# Autodesk Inventor assembly: Assembly6
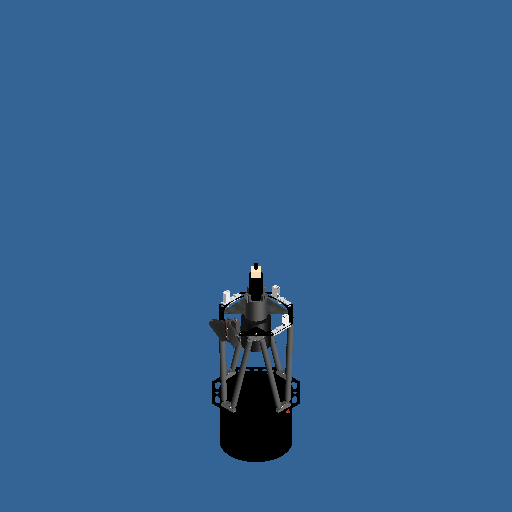
[picture p0: Inventor's stored thumbnail of the model, 512x512]
Saved by Autodesk Inventor 2026.2 (Build 302298000, 298)
## iProperties
Created: 2025-12-09
Part Number: Assembly6
Document SubType Name: Assembly
Designer: Thoma
Mass: 27295.5 g
Surface Area: 25498 cm^2
Volume: 10830.6 cm^3
Density: 2.52023 g/cm^3
Author: Thoma
## Documents named in this file (33)
- C:\Users\Thoma\OneDrive\Desktop\dir\telescope_cover\main\version_2\Main_v5.iam
- C:\Users\Thoma\OneDrive\Desktop\dir\telescope_cover\telescope\version_3\Telescope_End.ipt
- C:\Users\Thoma\OneDrive\Desktop\dir\telescope_cover\telescope\version_3\Triangle.ipt
- C:\Users\Thoma\OneDrive\Desktop\dir\telescope_cover\telescope\version_3\Triangle_Bracket_Top.ipt
- C:\Users\Thoma\OneDrive\Desktop\dir\telescope_cover\telescope\version_3\Carbon_Fibre.ipt
- C:\Users\Thoma\OneDrive\Desktop\dir\telescope_cover\telescope\version_3\5mm Screw.ipt
- C:\Users\Thoma\OneDrive\Desktop\dir\telescope_cover\telescope\version_3\35mm_bolt.ipt
- C:\Users\Thoma\OneDrive\Desktop\dir\telescope_cover\telescope\version_3\Triangle_Bracket_Bottom_MIR.ipt
- C:\Users\Thoma\OneDrive\Desktop\dir\telescope_cover\telescope\version_3\Telescope_Base.ipt
- C:\Users\Thoma\OneDrive\Desktop\dir\telescope_cover\telescope\version_3\Full_shaft_Simplify_3.ipt
- C:\Users\Thoma\OneDrive\Desktop\dir\telescope_cover\telescope\version_3\30mm_bolt.ipt
- C:\Users\Thoma\OneDrive\Desktop\dir\telescope_cover\telescope\version_3\Baffle.ipt
- C:\Users\Thoma\OneDrive\Desktop\dir\telescope_cover\telescope\version_3\Bottom_End_Top.ipt
- C:\Users\Thoma\OneDrive\Desktop\dir\telescope_cover\telescope\version_3\Laser.ipt
- C:\Users\Thoma\OneDrive\Desktop\dir\telescope_cover\cover\central_cover_v1.ipt
- C:\Users\Thoma\OneDrive\Desktop\dir\telescope_cover\cover\base_plate_v11.ipt
- C:\Users\Thoma\OneDrive\Desktop\dir\telescope_cover\cover\base_plate_bottom_v5.ipt
- C:\Users\Thoma\OneDrive\Documents\Inventor\Content Center Files\R2026\en-US\ISO 4035(2)\ISO 4035 - M4 - ISO.ipt
- C:\Users\Thoma\OneDrive\Desktop\dir\telescope_cover\servo\DSS-M15S Servo.ipt
- C:\Users\Thoma\OneDrive\Documents\Inventor\Content Center Files\R2026\en-US\ISO 4762(2)\ISO 4762 - M4 x 16ISO.ipt
- C:\Users\Thoma\OneDrive\Desktop\dir\telescope_cover\cover\pawn_v3.ipt
- C:\Users\Thoma\OneDrive\Documents\Inventor\Content Center Files\R2026\en-US\DIN 6796\DIN 6796 - 2.ipt
- C:\Users\Thoma\OneDrive\Documents\Inventor\Content Center Files\R2026\en-US\DIN 912\DIN 912 - M2 x 0.4 x 8 x 7.ipt
- C:\Users\Thoma\OneDrive\Documents\Inventor\Content Center Files\R2026\en-US\DIN 912\DIN 912 - M2 x 0.4 x 5 x 4.ipt
- C:\Users\Thoma\OneDrive\Desktop\dir\telescope_cover\cover\rod_v11.ipt
- C:\Users\Thoma\OneDrive\Documents\Inventor\Content Center Files\R2026\en-US\ISO 7092\ISO 7092 - ST 4 - 140 HV.ipt
- C:\Users\Thoma\OneDrive\Desktop\dir\telescope_cover\cover\Cover_Upper_v5.ipt
- C:\Users\Thoma\OneDrive\Desktop\dir\telescope_cover\cover\4mm_washer_1mm.ipt
- C:\Users\Thoma\OneDrive\Documents\Inventor\Content Center Files\R2026\en-US\ISO 4762(2)\ISO 4762 - M4 x 20ISO.ipt
- C:\Users\Thoma\OneDrive\Documents\Inventor\Content Center Files\R2026\en-US\ISO 4032(2)\ISO 4032 - M4 - ISO.ipt
- C:\Users\Thoma\OneDrive\Documents\Inventor\Content Center Files\R2026\en-US\ISO 7093 A\ISO 7093 A - ST 4 - 140 HV .ipt
- C:\Users\Thoma\OneDrive\Documents\Inventor\Content Center Files\R2026\en-US\ISO 4762(2)\ISO 4762 - M4 x 30ISO.ipt
- C:\Users\Thoma\OneDrive\Desktop\dir\telescope_cover\servo\limit_switch_v2.ipt
## Components (119 placed, 32 different names)
1. base_plate_bottom_v5:2 — Mate:332, Mate:333, Mate:334, Mate:353, Mate:357, Mate:361
2. base_plate_v11:2 — Mate:341, Mate:344, Mate:345
3. base_plate_bottom_v5:3 — Mate:338, Mate:339, Mate:340
4. base_plate_v11:3 — Mate:343, Mate:348, Mate:349, Mate:350, Mate:351, Mate:352, Mate:354, Mate:355, Mate:356, Mate:358, Mate:359, Mate:360
5. base_plate_bottom_v5:4 — Mate:335, Mate:336, Mate:337
6. base_plate_v11:4 — Mate:342, Mate:346, Mate:347
7. ISO 7092 ST 4 - 140 HV:14 — Mate:350, Mate:351, Insert:26
8. ISO 4762 M4 x 30:2 — Insert:26
9. ISO 7093 A ST 4 - 140 HV - A:4 — Mate:352, Mate:353, Insert:27
10. ISO 4032 M4:5 — Insert:27
11. ISO 7092 ST 4 - 140 HV:15 — Mate:354, Mate:355, Insert:28
12. ISO 4762 M4 x 20:6 — Insert:28
13. ISO 7093 A ST 4 - 140 HV - A:5 — Mate:356, Mate:357, Insert:29
14. ISO 4032 M4:6 — Insert:29
15. ISO 7092 ST 4 - 140 HV:16 — Mate:358, Mate:359, Insert:30
16. ISO 4762 M4 x 20:7 — Insert:30
17. ISO 7093 A ST 4 - 140 HV - A:6 — Mate:360, Mate:361, Insert:31
18. ISO 4032 M4:7 — Insert:31
19. base_plate_bottom_v5:5 — Mate:362, Mate:363, Mate:364, Mate:370, Mate:371, Flush:227
20. limit_switch_v2:1 — Mate:367, Mate:368, Mate:369
21. limit_switch_v2:2 — Mate:370, Mate:371, Flush:227
22. Laser:2 — Mate:214, Flush:220, Flush:221
23. Laser:1 — Mate:215, Flush:218, Flush:219
24. Baffle:1 — Mate:83
25. Carbon_Fibre:1 — Mate:7, Mate:11, Flush:1, Mate:12, Mate:13, Mate:14, Mate:15, Mate:62, Mate:83, Mate:92, Mate:93, Mate:96, Mate:97, Mate:98, Mate:100, Mate:123, Mate:124, Mate:125, Mate:213, Mate:220, Angle:84, Flush:223, Flush:224, Flush:225, Flush:226
26. Telescope_Base:1 — Mate:62, Angle:31, Mate:89, Mate:90, Angle:40, Mate:108, Mate:109, Angle:48, Mate:110, Mate:111, Angle:49, Mate:112, Mate:113, Angle:50, Mate:214, Mate:215, Flush:218, Flush:221
27. Telescope_End:1 — Mate:1, Mate:2, Angle:2, Mate:7, Mate:54, Mate:55, Angle:26, Angle:31, Mate:86, Mate:88, Mate:91, Angle:41, Mate:101, Angle:45, Angle:46, Mate:114, Mate:115, Angle:51, Mate:116, Mate:117, Angle:52, Mate:118, Mate:119, Angle:53, Mate:229, Angle:85, Mate:230, Mate:231, Mate:332, Mate:333, Mate:334, Mate:335, Mate:336, Mate:337, Mate:338, Mate:339, Mate:340, Mate:341, Mate:342, Mate:343, Mate:344, Mate:345, Mate:346, Mate:347, Mate:348, Mate:349, Mate:362
28. 30mm_bolt:9 — Mate:217, Mate:218, Angle:83
29. 30mm_bolt:10 — Mate:216, Mate:219, Angle:82
30. Triangle_Bracket_Top:5 — Mate:116, Mate:117, Angle:52, Mate:129, Flush:110, Angle:60
31. Triangle_Bracket_Top:4 — Mate:101, Angle:45, Angle:46, Mate:104, Mate:105, Mate:106, Flush:103, Angle:47
32. Triangle_Bracket_Top:3 — Mate:86, Mate:88, Mate:94, Angle:54, Angle:55, Mate:122, Flush:106, Angle:56
33. Triangle_Bracket_Top:1 — Mate:1, Mate:2, Angle:2, Mate:8, Mate:9, Angle:4, Mate:47, Angle:22, Mate:58
34. 5mm Screw:14 — Mate:220, Flush:222, Angle:84
35. Triangle:1 — Mate:8, Mate:9, Angle:4, Mate:11, Flush:1, Angle:5, Angle:6, Mate:46, Mate:222, Mate:223
36. Triangle:5 — Mate:92, Mate:93, Mate:94, Mate:128, Flush:109, Angle:59, Flush:181, Angle:81, Mate:225, Mate:227
37. Triangle:6 — Mate:96, Mate:97, Mate:98, Flush:102, Angle:44, Mate:104, Mate:105, Flush:222, Mate:221, Mate:228
38. Triangle:7 — Mate:123, Mate:124, Mate:125, Mate:126, Flush:107, Angle:57, Mate:127, Flush:108, Angle:58, Mate:224, Mate:226
39. 35mm_bolt:6 — Mate:122, Flush:106, Angle:56
40. 35mm_bolt:7 — Mate:129, Flush:110, Angle:60
41. 35mm_bolt:4 — Mate:46, Mate:47, Angle:22
42. 35mm_bolt:5 — Mate:106, Flush:103, Angle:47
43. 5mm Screw:9 — Mate:100, Flush:102, Angle:44
44. 5mm Screw:13 — Mate:213, Flush:181, Angle:81
45. 5mm Screw:10 — Mate:126, Flush:107, Angle:57
46. 5mm Screw:2 — Mate:14, Mate:15, Angle:6
47. 5mm Screw:1 — Mate:12, Mate:13, Angle:5
48. 5mm Screw:11 — Mate:127, Flush:108, Angle:58
49. 5mm Screw:12 — Mate:128, Flush:109, Angle:59
50. Full_shaft_Simplify_3:1
51. Full_shaft_Simplify_3:2 — Tangent:26
52. Full_shaft_Simplify_3:3
53. Full_shaft_Simplify_3:4
54. Full_shaft_Simplify_3:5
55. Full_shaft_Simplify_3:6
56. Full_shaft_Simplify_3:7
57. Full_shaft_Simplify_3:8 — Tangent:31, Tangent:33
58. 30mm_bolt:7 — Mate:120, Flush:104, Angle:54
59. 30mm_bolt:1 — Mate:121, Flush:105, Angle:55
60. 30mm_bolt:8 — Mate:80, Flush:13, Angle:39
61. 30mm_bolt:6 — Mate:78, Flush:11, Angle:37
62. 30mm_bolt:3 — Mate:79, Flush:12, Angle:38
63. 30mm_bolt:2 — Mate:77, Flush:10, Angle:36
64. Triangle_Bracket_Bottom_MIR:4 — Mate:118, Mate:119, Angle:53, Mate:216, Mate:217, Mate:218, Mate:219, Angle:82, Angle:83
65. Triangle_Bracket_Bottom_MIR:3 — Mate:114, Mate:115, Angle:51, Mate:120, Flush:104, Mate:121, Flush:105
66. Triangle_Bracket_Bottom_MIR:2 — Mate:55, Mate:58, Angle:26, Mate:77, Flush:10, Angle:36, Mate:78, Flush:11, Angle:37, Tangent:31
67. Triangle_Bracket_Bottom_MIR:1 — Mate:54, Mate:79, Flush:12, Angle:38, Mate:80, Flush:13, Angle:39, Mate:91, Angle:41
68. Bottom_End_Top:4 — Mate:112, Mate:113, Angle:50, Tangent:26, Tangent:33
69. Bottom_End_Top:3 — Mate:110, Mate:111, Angle:49, Flush:219
70. Bottom_End_Top:2 — Mate:108, Mate:109, Angle:48
71. Bottom_End_Top:1 — Mate:89, Mate:90, Angle:40, Flush:220
72. central_cover_v1:1 — Mate:221, Mate:222, Flush:223, Mate:367, Mate:368, Mate:369
73. central_cover_v1:2 — Mate:223, Mate:224, Flush:224
74. central_cover_v1:3 — Mate:225, Mate:226, Flush:225
75. central_cover_v1:4 — Mate:227, Mate:228, Flush:226
76. base_plate_v11:1 — Mate:229, Angle:85, Mate:230, Mate:231, Angle:92, Mate:262, Mate:263, Mate:264, Mate:271, Mate:272, Mate:273, Mate:274, Mate:275, Mate:276, Mate:277, Mate:278, Mate:282, Mate:307, Mate:308, Mate:309, Mate:310, Mate:312, Mate:314, Mate:320, Mate:321, Mate:322, Mate:324, Mate:325, Mate:326, Mate:328, Mate:329, Mate:330
77. pawn_v3:1 — Angle:92, Mate:281, Mate:282, Mate:311, Mate:313
78. DSS-M15S Servo:1 — Mate:262, Mate:263, Mate:264, Mate:279, Mate:280
79. DIN 6796 2:1 — Mate:271, Mate:272, Insert:6
80. DIN 912 - replaced by DIN EN ISO 4762 M2 x 8:1 — Insert:6
81. DIN 6796 2:2 — Mate:273, Mate:274, Insert:7
82. DIN 912 - replaced by DIN EN ISO 4762 M2 x 5:1 — Insert:7
83. DIN 6796 2:3 — Mate:275, Mate:276, Insert:8
84. DIN 912 - replaced by DIN EN ISO 4762 M2 x 8:2 — Insert:8
85. DIN 6796 2:4 — Mate:277, Mate:278, Insert:9
86. DIN 912 - replaced by DIN EN ISO 4762 M2 x 8:3 — Insert:9
87. rod_v11:1 — Mate:279, Mate:280, Mate:281, Mate:287, Mate:288, Tangent:34, Mate:289, Mate:290, Mate:291, Mate:292, Mate:293, Mate:294, Mate:295, Mate:297, Mate:298, Mate:299, Mate:301, Mate:302, Mate:303, Mate:305, Mate:306
88. Cover_Upper_v5:1 — Mate:287, Mate:288, Tangent:34, Mate:296, Mate:300, Mate:304
89. 4mm_washer_1mm:1 — Mate:289, Mate:294
90. 4mm_washer_1mm:2 — Mate:290, Mate:293
91. 4mm_washer_1mm:3 — Mate:291, Mate:292
92. ISO 7092 ST 4 - 140 HV:3 — Mate:295, Mate:296, Insert:12
93. ISO 4762 M4 x 16:3 — Insert:12
94. ISO 7092 ST 4 - 140 HV:4 — Mate:297, Mate:298, Insert:13
95. ISO 4035 M4:5 — Insert:13
96. ISO 7092 ST 4 - 140 HV:5 — Mate:299, Mate:300, Insert:14
97. ISO 4762 M4 x 16:4 — Insert:14
98. ISO 7092 ST 4 - 140 HV:6 — Mate:301, Mate:302, Insert:15
99. ISO 4035 M4:6 — Insert:15
100. ISO 7092 ST 4 - 140 HV:7 — Mate:303, Mate:304, Insert:16
101. ISO 4762 M4 x 16:5 — Insert:16
102. ISO 7092 ST 4 - 140 HV:8 — Mate:305, Mate:306, Insert:17
103. ISO 4035 M4:7 — Insert:17
104. ISO 4762 M4 x 20:1 — Mate:307, Mate:308
105. ISO 4035 M4:8 — Mate:309, Mate:310
106. ISO 4762 M4 x 20:2 — Mate:311, Mate:312
107. ISO 4035 M4:9 — Mate:313, Mate:314
108. ISO 7092 ST 4 - 140 HV:11 — Mate:320, Mate:321, Insert:20
109. ISO 4762 M4 x 20:4 — Insert:20
110. ISO 7093 A ST 4 - 140 HV - A:1 — Mate:322, Insert:21
111. ISO 4032 M4:2 — Insert:21
112. ISO 7092 ST 4 - 140 HV:12 — Mate:324, Mate:325, Insert:22
113. ISO 4762 M4 x 20:5 — Insert:22, Mate:363
114. ISO 7093 A ST 4 - 140 HV - A:2 — Mate:326, Insert:23
115. ISO 4032 M4:3 — Insert:23
116. ISO 7092 ST 4 - 140 HV:13 — Mate:328, Mate:329, Insert:24
117. ISO 4762 M4 x 30:1 — Insert:24, Mate:364
118. ISO 7093 A ST 4 - 140 HV - A:3 — Mate:330, Insert:25
119. ISO 4032 M4:4 — Insert:25
## Relationships (255: Mate 168, Angle 36, Flush 25, Insert 22, Tangent 4)
- Mate:1: Telescope_End:1 ↔ Triangle_Bracket_Top:1
- Mate:2: Telescope_End:1 ↔ Triangle_Bracket_Top:1
- Angle:2 (0 deg): Telescope_End:1 ↔ Triangle_Bracket_Top:1
- Mate:7: Carbon_Fibre:1 ↔ Telescope_End:1
- Mate:8: Triangle_Bracket_Top:1 ↔ Triangle:1
- Mate:9: Triangle_Bracket_Top:1 ↔ Triangle:1
- Angle:4 (0 deg): Triangle_Bracket_Top:1 ↔ Triangle:1
- Mate:11: Carbon_Fibre:1 ↔ Triangle:1
- Flush:1: Carbon_Fibre:1 ↔ Triangle:1
- Mate:12: Carbon_Fibre:1 ↔ 5mm Screw:1
- Mate:13: Carbon_Fibre:1 ↔ 5mm Screw:1
- Angle:5 (0 deg): Triangle:1 ↔ 5mm Screw:1
- Mate:14: Carbon_Fibre:1 ↔ 5mm Screw:2
- Mate:15: Carbon_Fibre:1 ↔ 5mm Screw:2
- Angle:6 (0 deg): Triangle:1 ↔ 5mm Screw:2
- Mate:46: Triangle:1 ↔ 35mm_bolt:4
- Mate:47: Triangle_Bracket_Top:1 ↔ 35mm_bolt:4
- Angle:22 (0 deg): Triangle_Bracket_Top:1 ↔ 35mm_bolt:4
- Mate:54: Telescope_End:1 ↔ Triangle_Bracket_Bottom_MIR:1
- Mate:55: Telescope_End:1 ↔ Triangle_Bracket_Bottom_MIR:2
- Mate:58: Triangle_Bracket_Top:1 ↔ Triangle_Bracket_Bottom_MIR:2
- Angle:26 (0 deg): Telescope_End:1 ↔ Triangle_Bracket_Bottom_MIR:2
- Mate:62: Carbon_Fibre:1 ↔ Telescope_Base:1
- Angle:31 (0 deg): Telescope_Base:1 ↔ Telescope_End:1
- Mate:77: 30mm_bolt:2 ↔ Triangle_Bracket_Bottom_MIR:2
- Flush:10: 30mm_bolt:2 ↔ Triangle_Bracket_Bottom_MIR:2
- Angle:36 (0 deg): 30mm_bolt:2 ↔ Triangle_Bracket_Bottom_MIR:2
- Mate:78: 30mm_bolt:6 ↔ Triangle_Bracket_Bottom_MIR:2
- Flush:11: 30mm_bolt:6 ↔ Triangle_Bracket_Bottom_MIR:2
- Angle:37 (0 deg): 30mm_bolt:6 ↔ Triangle_Bracket_Bottom_MIR:2
- Mate:79: 30mm_bolt:3 ↔ Triangle_Bracket_Bottom_MIR:1
- Flush:12: 30mm_bolt:3 ↔ Triangle_Bracket_Bottom_MIR:1
- Angle:38 (0 deg): 30mm_bolt:3 ↔ Triangle_Bracket_Bottom_MIR:1
- Mate:80: 30mm_bolt:8 ↔ Triangle_Bracket_Bottom_MIR:1
- Flush:13: 30mm_bolt:8 ↔ Triangle_Bracket_Bottom_MIR:1
- Angle:39 (0 deg): 30mm_bolt:8 ↔ Triangle_Bracket_Bottom_MIR:1
- Mate:83: Baffle:1 ↔ Carbon_Fibre:1
- Mate:86: Telescope_End:1 ↔ Triangle_Bracket_Top:3
- Mate:88: Telescope_End:1 ↔ Triangle_Bracket_Top:3
- Mate:89: Telescope_Base:1 ↔ Bottom_End_Top:1
- Mate:90: Telescope_Base:1 ↔ Bottom_End_Top:1
- Angle:40 (0 deg): Telescope_Base:1 ↔ Bottom_End_Top:1
- Mate:91: Telescope_End:1 ↔ Triangle_Bracket_Bottom_MIR:1
- Angle:41 (0 deg): Telescope_End:1 ↔ Triangle_Bracket_Bottom_MIR:1
- Mate:92: Carbon_Fibre:1 ↔ Triangle:5
- Mate:93: Carbon_Fibre:1 ↔ Triangle:5
- Mate:94: Triangle_Bracket_Top:3 ↔ Triangle:5
- Mate:96: Carbon_Fibre:1 ↔ Triangle:6
- Mate:97: Carbon_Fibre:1 ↔ Triangle:6
- Mate:98: Carbon_Fibre:1 ↔ Triangle:6
- Mate:100: Carbon_Fibre:1 ↔ 5mm Screw:9
- Flush:102: Triangle:6 ↔ 5mm Screw:9
- Angle:44 (0 deg): Triangle:6 ↔ 5mm Screw:9
- Mate:101: Telescope_End:1 ↔ Triangle_Bracket_Top:4
- Angle:45 (0 deg): Telescope_End:1 ↔ Triangle_Bracket_Top:4
- Angle:46 (0 deg): Telescope_End:1 ↔ Triangle_Bracket_Top:4
- Mate:104: Triangle_Bracket_Top:4 ↔ Triangle:6
- Mate:105: Triangle_Bracket_Top:4 ↔ Triangle:6
- Mate:106: Triangle_Bracket_Top:4 ↔ 35mm_bolt:5
- Flush:103: Triangle_Bracket_Top:4 ↔ 35mm_bolt:5
- Angle:47 (0 deg): Triangle_Bracket_Top:4 ↔ 35mm_bolt:5
- Mate:108: Telescope_Base:1 ↔ Bottom_End_Top:2
- Mate:109: Telescope_Base:1 ↔ Bottom_End_Top:2
- Angle:48 (0 deg): Telescope_Base:1 ↔ Bottom_End_Top:2
- Mate:110: Telescope_Base:1 ↔ Bottom_End_Top:3
- Mate:111: Telescope_Base:1 ↔ Bottom_End_Top:3
- Angle:49 (0 deg): Telescope_Base:1 ↔ Bottom_End_Top:3
- Mate:112: Telescope_Base:1 ↔ Bottom_End_Top:4
- Mate:113: Telescope_Base:1 ↔ Bottom_End_Top:4
- Angle:50 (0 deg): Telescope_Base:1 ↔ Bottom_End_Top:4
- Mate:114: Telescope_End:1 ↔ Triangle_Bracket_Bottom_MIR:3
- Mate:115: Telescope_End:1 ↔ Triangle_Bracket_Bottom_MIR:3
- Angle:51 (0 deg): Telescope_End:1 ↔ Triangle_Bracket_Bottom_MIR:3
- Mate:116: Telescope_End:1 ↔ Triangle_Bracket_Top:5
- Mate:117: Telescope_End:1 ↔ Triangle_Bracket_Top:5
- Angle:52 (0 deg): Telescope_End:1 ↔ Triangle_Bracket_Top:5
- Mate:118: Telescope_End:1 ↔ Triangle_Bracket_Bottom_MIR:4
- Mate:119: Telescope_End:1 ↔ Triangle_Bracket_Bottom_MIR:4
- Angle:53 (0 deg): Telescope_End:1 ↔ Triangle_Bracket_Bottom_MIR:4
- Mate:120: 30mm_bolt:7 ↔ Triangle_Bracket_Bottom_MIR:3
- Flush:104: 30mm_bolt:7 ↔ Triangle_Bracket_Bottom_MIR:3
- Angle:54 (0 deg): Triangle_Bracket_Top:3 ↔ 30mm_bolt:7
- Mate:121: 30mm_bolt:1 ↔ Triangle_Bracket_Bottom_MIR:3
- Flush:105: 30mm_bolt:1 ↔ Triangle_Bracket_Bottom_MIR:3
- Angle:55 (0 deg): Triangle_Bracket_Top:3 ↔ 30mm_bolt:1
- Mate:122: Triangle_Bracket_Top:3 ↔ 35mm_bolt:6
- Flush:106: Triangle_Bracket_Top:3 ↔ 35mm_bolt:6
- Angle:56 (0 deg): Triangle_Bracket_Top:3 ↔ 35mm_bolt:6
- Mate:123: Carbon_Fibre:1 ↔ Triangle:7
- Mate:124: Carbon_Fibre:1 ↔ Triangle:7
- Mate:125: Carbon_Fibre:1 ↔ Triangle:7
- Mate:126: Triangle:7 ↔ 5mm Screw:10
- Flush:107: Triangle:7 ↔ 5mm Screw:10
- Angle:57 (0 deg): Triangle:7 ↔ 5mm Screw:10
- Mate:127: Triangle:7 ↔ 5mm Screw:11
- Flush:108: Triangle:7 ↔ 5mm Screw:11
- Angle:58 (0 deg): Triangle:7 ↔ 5mm Screw:11
- Mate:128: Triangle:5 ↔ 5mm Screw:12
- Flush:109: Triangle:5 ↔ 5mm Screw:12
- Angle:59 (0 deg): Triangle:5 ↔ 5mm Screw:12
- Mate:129: Triangle_Bracket_Top:5 ↔ 35mm_bolt:7
- Flush:110: Triangle_Bracket_Top:5 ↔ 35mm_bolt:7
- Angle:60 (0 deg): Triangle_Bracket_Top:5 ↔ 35mm_bolt:7
- Mate:213: Carbon_Fibre:1 ↔ 5mm Screw:13
- Flush:181: Triangle:5 ↔ 5mm Screw:13
- Angle:81 (0 deg): Triangle:5 ↔ 5mm Screw:13
- Mate:214: Laser:2 ↔ Telescope_Base:1
- Mate:215: Laser:1 ↔ Telescope_Base:1
- Flush:218: Laser:1 ↔ Telescope_Base:1
- Flush:219 (39.316 mm): Laser:1 ↔ Bottom_End_Top:3
- Flush:220 (39.316 mm): Laser:2 ↔ Bottom_End_Top:1
- Flush:221: Laser:2 ↔ Telescope_Base:1
- Tangent:26: Full_shaft_Simplify_3:2 ↔ Bottom_End_Top:4
- Tangent:31: Full_shaft_Simplify_3:8 ↔ Triangle_Bracket_Bottom_MIR:2
- Tangent:33: Full_shaft_Simplify_3:8 ↔ Bottom_End_Top:4
- Mate:216: 30mm_bolt:10 ↔ Triangle_Bracket_Bottom_MIR:4
- Mate:217: 30mm_bolt:9 ↔ Triangle_Bracket_Bottom_MIR:4
- Mate:218: 30mm_bolt:9 ↔ Triangle_Bracket_Bottom_MIR:4
- Mate:219: 30mm_bolt:10 ↔ Triangle_Bracket_Bottom_MIR:4
- Angle:82 (0 deg): 30mm_bolt:10 ↔ Triangle_Bracket_Bottom_MIR:4
- Angle:83 (0 deg): 30mm_bolt:9 ↔ Triangle_Bracket_Bottom_MIR:4
- Mate:220: Carbon_Fibre:1 ↔ 5mm Screw:14
- Flush:222: 5mm Screw:14 ↔ Triangle:6
- Angle:84 (0 deg): Carbon_Fibre:1 ↔ 5mm Screw:14
- Mate:221: Triangle:6 ↔ central_cover_v1:1
- Mate:222: Triangle:1 ↔ central_cover_v1:1
- Flush:223: Carbon_Fibre:1 ↔ central_cover_v1:1
- Mate:223: Triangle:1 ↔ central_cover_v1:2
- Mate:224: Triangle:7 ↔ central_cover_v1:2
- Flush:224: Carbon_Fibre:1 ↔ central_cover_v1:2
- Mate:225: Triangle:5 ↔ central_cover_v1:3
- Mate:226: Triangle:7 ↔ central_cover_v1:3
- Flush:225: Carbon_Fibre:1 ↔ central_cover_v1:3
- Mate:227: Triangle:5 ↔ central_cover_v1:4
- Mate:228: Triangle:6 ↔ central_cover_v1:4
- Flush:226: Carbon_Fibre:1 ↔ central_cover_v1:4
- Mate:229: Telescope_End:1 ↔ base_plate_v11:1
- Angle:85 (0 deg): Telescope_End:1 ↔ base_plate_v11:1
- Mate:230: Telescope_End:1 ↔ base_plate_v11:1
- Mate:231: Telescope_End:1 ↔ base_plate_v11:1
- Angle:92 (0 deg): base_plate_v11:1 ↔ pawn_v3:1
- Mate:262: base_plate_v11:1 ↔ DSS-M15S Servo:1
- Mate:263 (1.1 mm): base_plate_v11:1 ↔ DSS-M15S Servo:1
- Mate:264: base_plate_v11:1 ↔ DSS-M15S Servo:1
- Mate:271: base_plate_v11:1 ↔ DIN 6796 2:1
- Mate:272: base_plate_v11:1 ↔ DIN 6796 2:1
- Insert:6: DIN 6796 2:1 ↔ DIN 912 - replaced by DIN EN ISO 4762 M2 x 8:1
- Mate:273: base_plate_v11:1 ↔ DIN 6796 2:2
- Mate:274: base_plate_v11:1 ↔ DIN 6796 2:2
- Insert:7: DIN 6796 2:2 ↔ DIN 912 - replaced by DIN EN ISO 4762 M2 x 5:1
- Mate:275: base_plate_v11:1 ↔ DIN 6796 2:3
- Mate:276: base_plate_v11:1 ↔ DIN 6796 2:3
- Insert:8: DIN 6796 2:3 ↔ DIN 912 - replaced by DIN EN ISO 4762 M2 x 8:2
- Mate:277: base_plate_v11:1 ↔ DIN 6796 2:4
- Mate:278: base_plate_v11:1 ↔ DIN 6796 2:4
- Insert:9: DIN 6796 2:4 ↔ DIN 912 - replaced by DIN EN ISO 4762 M2 x 8:3
- Mate:279: DSS-M15S Servo:1 ↔ rod_v11:1
- Mate:280: DSS-M15S Servo:1 ↔ rod_v11:1
- Mate:281: pawn_v3:1 ↔ rod_v11:1
- Mate:282 (0.4 mm): base_plate_v11:1 ↔ pawn_v3:1
- Mate:287: rod_v11:1 ↔ Cover_Upper_v5:1
- Mate:288: rod_v11:1 ↔ Cover_Upper_v5:1
- Tangent:34 (-1 mm): rod_v11:1 ↔ Cover_Upper_v5:1
- Mate:289: rod_v11:1 ↔ 4mm_washer_1mm:1
- Mate:290: rod_v11:1 ↔ 4mm_washer_1mm:2
- Mate:291: rod_v11:1 ↔ 4mm_washer_1mm:3
- Mate:292: rod_v11:1 ↔ 4mm_washer_1mm:3
- Mate:293: rod_v11:1 ↔ 4mm_washer_1mm:2
- Mate:294: rod_v11:1 ↔ 4mm_washer_1mm:1
- Mate:295: rod_v11:1 ↔ ISO 7092 ST 4 - 140 HV:3
- Mate:296: Cover_Upper_v5:1 ↔ ISO 7092 ST 4 - 140 HV:3
- Insert:12: ISO 7092 ST 4 - 140 HV:3 ↔ ISO 4762 M4 x 16:3
- Mate:297: rod_v11:1 ↔ ISO 7092 ST 4 - 140 HV:4
- Mate:298: rod_v11:1 ↔ ISO 7092 ST 4 - 140 HV:4
- Insert:13: ISO 7092 ST 4 - 140 HV:4 ↔ ISO 4035 M4:5
- Mate:299: rod_v11:1 ↔ ISO 7092 ST 4 - 140 HV:5
- Mate:300: Cover_Upper_v5:1 ↔ ISO 7092 ST 4 - 140 HV:5
- Insert:14: ISO 7092 ST 4 - 140 HV:5 ↔ ISO 4762 M4 x 16:4
- Mate:301: rod_v11:1 ↔ ISO 7092 ST 4 - 140 HV:6
- Mate:302: rod_v11:1 ↔ ISO 7092 ST 4 - 140 HV:6
- Insert:15: ISO 7092 ST 4 - 140 HV:6 ↔ ISO 4035 M4:6
- Mate:303: rod_v11:1 ↔ ISO 7092 ST 4 - 140 HV:7
- Mate:304: Cover_Upper_v5:1 ↔ ISO 7092 ST 4 - 140 HV:7
- Insert:16: ISO 7092 ST 4 - 140 HV:7 ↔ ISO 4762 M4 x 16:5
- Mate:305: rod_v11:1 ↔ ISO 7092 ST 4 - 140 HV:8
- Mate:306: rod_v11:1 ↔ ISO 7092 ST 4 - 140 HV:8
- Insert:17: ISO 7092 ST 4 - 140 HV:8 ↔ ISO 4035 M4:7
- Mate:307: base_plate_v11:1 ↔ ISO 4762 M4 x 20:1
- Mate:308: base_plate_v11:1 ↔ ISO 4762 M4 x 20:1
- Mate:309: base_plate_v11:1 ↔ ISO 4035 M4:8
- Mate:310: base_plate_v11:1 ↔ ISO 4035 M4:8
- Mate:311: pawn_v3:1 ↔ ISO 4762 M4 x 20:2
- Mate:312: base_plate_v11:1 ↔ ISO 4762 M4 x 20:2
- Mate:313: pawn_v3:1 ↔ ISO 4035 M4:9
- Mate:314: base_plate_v11:1 ↔ ISO 4035 M4:9
- Mate:320: base_plate_v11:1 ↔ ISO 7092 ST 4 - 140 HV:11
- Mate:321: base_plate_v11:1 ↔ ISO 7092 ST 4 - 140 HV:11
- Insert:20: ISO 7092 ST 4 - 140 HV:11 ↔ ISO 4762 M4 x 20:4
- Mate:322: base_plate_v11:1 ↔ ISO 7093 A ST 4 - 140 HV - A:1
- Insert:21: ISO 7093 A ST 4 - 140 HV - A:1 ↔ ISO 4032 M4:2
- Mate:324: base_plate_v11:1 ↔ ISO 7092 ST 4 - 140 HV:12
- Mate:325: base_plate_v11:1 ↔ ISO 7092 ST 4 - 140 HV:12
- Insert:22: ISO 7092 ST 4 - 140 HV:12 ↔ ISO 4762 M4 x 20:5
- Mate:326: base_plate_v11:1 ↔ ISO 7093 A ST 4 - 140 HV - A:2
- Insert:23: ISO 7093 A ST 4 - 140 HV - A:2 ↔ ISO 4032 M4:3
- Mate:328: base_plate_v11:1 ↔ ISO 7092 ST 4 - 140 HV:13
- Mate:329: base_plate_v11:1 ↔ ISO 7092 ST 4 - 140 HV:13
- Insert:24: ISO 7092 ST 4 - 140 HV:13 ↔ ISO 4762 M4 x 30:1
- Mate:330: base_plate_v11:1 ↔ ISO 7093 A ST 4 - 140 HV - A:3
- Insert:25: ISO 7093 A ST 4 - 140 HV - A:3 ↔ ISO 4032 M4:4
- Mate:332: base_plate_bottom_v5:2 ↔ Telescope_End:1
- Mate:333: base_plate_bottom_v5:2 ↔ Telescope_End:1
- Mate:334: base_plate_bottom_v5:2 ↔ Telescope_End:1
- Mate:335: base_plate_bottom_v5:4 ↔ Telescope_End:1
- Mate:336: base_plate_bottom_v5:4 ↔ Telescope_End:1
- Mate:337: base_plate_bottom_v5:4 ↔ Telescope_End:1
- Mate:338: base_plate_bottom_v5:3 ↔ Telescope_End:1
- Mate:339: base_plate_bottom_v5:3 ↔ Telescope_End:1
- Mate:340: base_plate_bottom_v5:3 ↔ Telescope_End:1
- Mate:341: base_plate_v11:2 ↔ Telescope_End:1
- Mate:342: base_plate_v11:4 ↔ Telescope_End:1
- Mate:343: base_plate_v11:3 ↔ Telescope_End:1
- Mate:344: base_plate_v11:2 ↔ Telescope_End:1
- Mate:345: base_plate_v11:2 ↔ Telescope_End:1
- Mate:346: base_plate_v11:4 ↔ Telescope_End:1
- Mate:347: base_plate_v11:4 ↔ Telescope_End:1
- Mate:348: base_plate_v11:3 ↔ Telescope_End:1
- Mate:349: base_plate_v11:3 ↔ Telescope_End:1
- Mate:350: base_plate_v11:3 ↔ ISO 7092 ST 4 - 140 HV:14
- Mate:351: base_plate_v11:3 ↔ ISO 7092 ST 4 - 140 HV:14
- Insert:26: ISO 7092 ST 4 - 140 HV:14 ↔ ISO 4762 M4 x 30:2
- Mate:352: base_plate_v11:3 ↔ ISO 7093 A ST 4 - 140 HV - A:4
- Mate:353: base_plate_bottom_v5:2 ↔ ISO 7093 A ST 4 - 140 HV - A:4
- Insert:27: ISO 7093 A ST 4 - 140 HV - A:4 ↔ ISO 4032 M4:5
- Mate:354: base_plate_v11:3 ↔ ISO 7092 ST 4 - 140 HV:15
- Mate:355: base_plate_v11:3 ↔ ISO 7092 ST 4 - 140 HV:15
- Insert:28: ISO 7092 ST 4 - 140 HV:15 ↔ ISO 4762 M4 x 20:6
- Mate:356: base_plate_v11:3 ↔ ISO 7093 A ST 4 - 140 HV - A:5
- Mate:357: base_plate_bottom_v5:2 ↔ ISO 7093 A ST 4 - 140 HV - A:5
- Insert:29: ISO 7093 A ST 4 - 140 HV - A:5 ↔ ISO 4032 M4:6
- Mate:358: base_plate_v11:3 ↔ ISO 7092 ST 4 - 140 HV:16
- Mate:359: base_plate_v11:3 ↔ ISO 7092 ST 4 - 140 HV:16
- Insert:30: ISO 7092 ST 4 - 140 HV:16 ↔ ISO 4762 M4 x 20:7
- Mate:360: base_plate_v11:3 ↔ ISO 7093 A ST 4 - 140 HV - A:6
- Mate:361: base_plate_bottom_v5:2 ↔ ISO 7093 A ST 4 - 140 HV - A:6
- Insert:31: ISO 7093 A ST 4 - 140 HV - A:6 ↔ ISO 4032 M4:7
- Mate:362: base_plate_bottom_v5:5 ↔ Telescope_End:1
- Mate:363: base_plate_bottom_v5:5 ↔ ISO 4762 M4 x 20:5
- Mate:364: base_plate_bottom_v5:5 ↔ ISO 4762 M4 x 30:1
- Mate:367 (0.4 mm): limit_switch_v2:1 ↔ central_cover_v1:1
- Mate:368 (0.4 mm): limit_switch_v2:1 ↔ central_cover_v1:1
- Mate:369 (-17.1 mm): limit_switch_v2:1 ↔ central_cover_v1:1
- Mate:370 (0.4 mm): base_plate_bottom_v5:5 ↔ limit_switch_v2:2
- Mate:371 (0.4 mm): base_plate_bottom_v5:5 ↔ limit_switch_v2:2
- Flush:227: base_plate_bottom_v5:5 ↔ limit_switch_v2:2
